# Autodesk Inventor assembly: Ensemble1
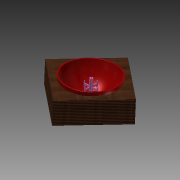
[picture p0: Inventor's stored thumbnail of the model, 180x180]
Saved by Autodesk Inventor 2015 (Build 190159000, 159)
## iProperties
Created: 2019-02-09
Part Number: Ensemble1
Document SubType Name: Assembly
Designer: Naly jérémie
Author: Naly jérémie
## Documents named in this file (4)
- C:\Users\Naly jérémie\Documents\Arduino\Modelisation\Ensemble1.iam
- C:\Users\Naly jérémie\Documents\Arduino\Modelisation\Pièce1.ipt
- C:\Users\Naly jérémie\Documents\Arduino\Modelisation\Pièce2.ipt
- C:\Users\Naly jérémie\Documents\Arduino\Modelisation\Pièce3.ipt
## Components (3 placed, 3 different names)
1. Pièce1:1 — Placage:1, Tangente:1
2. Pièce2:1 — Placage:1, Tangente:1, Placage:2
3. Pièce3:1 — Placage:2
## Relationships (3: Mate 2, Tangent 1)
- Placage:1 [Mate]: Pièce1:1 ↔ Pièce2:1
- Tangente:1: Pièce1:1 ↔ Pièce2:1
- Placage:2 [Mate]: Pièce2:1 ↔ Pièce3:1
